# Autodesk Inventor assembly: Rover
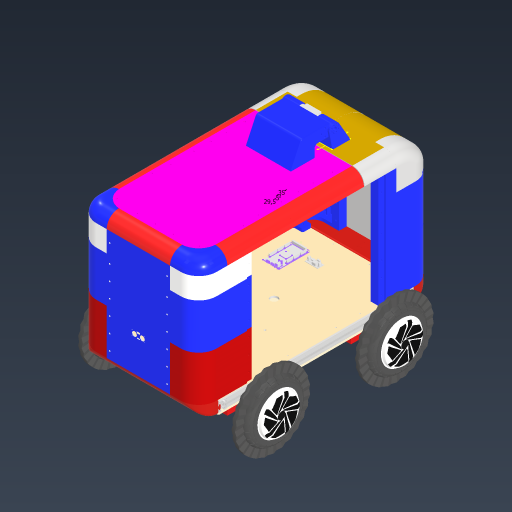
[picture p0: Inventor's stored thumbnail of the model, 512x512]
Saved by Autodesk Inventor 2023.2 (Build 272271030, 271C)
## iProperties
Created: 2024-10-30
Part Number: Rover
Document SubType Name: Assembly
Designer: I9232
Author: I9232
## Documents named in this file (30)
- D:\!Rover\Rover\Rover_construction\Rover.iam
- D:\!Rover\Rover\Rover_construction\platform.ipt
- D:\!Rover\Rover\Rover_construction\Motor, BLDC, Hoverboard Wheel, 8.0in.ipt
- D:\!Rover\Rover\Rover_construction\Profil 20x20.ipt
- D:\!Rover\Rover\Rover_construction\Крепление мотора.iam
- D:\!Rover\Rover\Rover_construction\Уголок для профиля.ipt
- D:\!Rover\Rover\Rover_construction\Профиль 30x30\Профиль 30x30.ipt
- D:\!Rover\Rover\Rover_construction\Т-образный соединитель\Т-образный соединитель.ipt
- D:\!Rover\Rover\Rover_construction\Подъёмник.iam
- D:\!Rover\Rover\Rover_construction\Боковая часть корпуса.ipt
- D:\!Rover\Rover\Rover_construction\Передняя_Задняя фанера.ipt
- D:\!Rover\Rover\Rover_construction\Столбик.ipt
- D:\!Rover\Rover\Rover_construction\Крышка.ipt
- D:\!Rover\Rover\Rover_construction\Вторая часть петли.ipt
- D:\!Rover\Rover\Rover_construction\рдс150.ipt
- D:\!Rover\Rover\Rover_construction\Arduino_Due\Arduino_Due.ipt
- D:\!Rover\Rover\Rover_construction\LM2596 DC-DC stepdown voltage converter\LM2596 DC-DC stepdown voltage converter.ipt
- D:\!Rover\Rover\Rover_construction\DS51_Arm_Disc\DS51_Arm_Disc.ipt
- D:\!Rover\Rover\Rover_construction\Крепление датчика ульразвука.iam
- D:\!Rover\Rover\Rover_construction\Нижний край корпуса.ipt
- D:\!Rover\Rover\Rover_construction\Задний_столб.iam
- D:\!Rover\Rover\Rover_construction\Столб_переда_корпуса_2.0.iam
- D:\!Rover\Rover\Rover_construction\2.0_Ушко петли крышки.ipt
- D:\!Rover\Rover\Rover_construction\2.0_Ушко петли крышки_MIR.ipt
- D:\!Rover\Rover\Rover_construction\2.0_Уголок_передней_крышки.ipt
- D:\!Rover\Rover\Rover_construction\2.0_Уголок_передней_крышки_MIR.ipt
- D:\!Rover\Rover\Rover_construction\2.0_передняя_фанера.ipt
- D:\!Rover\Rover\Rover_construction\Столб_переда_корпуса_2.0_MIR1.iam
- D:\!Rover\Rover\Rover_construction\Задний_столб_MIR1.iam
- D:\!Rover\Rover\Rover_construction\Крышка.iam
## Components (51 placed, 29 different names)
1. platform:1 — Совмещение:1, Совмещение:2, Совмещение:169, Заподлицо:1, Заподлицо:2, Совмещение:170, Совмещение:171, Совмещение:172, Заподлицо:3, Заподлицо:4, Заподлицо:5, Заподлицо:6, Совмещение:180, Заподлицо:11, Совмещение:189, Заподлицо:24, Заподлицо:25, Совмещение:190, Заподлицо:26, Заподлицо:27, Заподлицо:28, Совмещение:191, Заподлицо:29, Совмещение:192, Заподлицо:30, Заподлицо:31, Заподлицо:37, Заподлицо:63
2. Т-образный соединитель:1 — Заподлицо:21, Совмещение:188
3. Т-образный соединитель:2 — Совмещение:187, Заподлицо:23
4. Подъёмник:1 [sub-assembly] — Совмещение:355, Совмещение:356
5. platform:2 — Заподлицо:37, Заподлицо:38, Совмещение:313, Совмещение:314, Совмещение:315, Совмещение:316, Совмещение:317, Заподлицо:46, Заподлицо:47, Совмещение:350, Совмещение:351, Совмещение:355, Заподлицо:62, Заподлицо:72
6. Боковая часть корпуса:1 — Симметрия:4
7. Боковая часть корпуса:2 — Симметрия:4
8. Передняя_Задняя фанера:2 — Совмещение:445, Совмещение:446, Совмещение:447, Совмещение:450
9. Столбик:2 — Совмещение:329, Заподлицо:46, Заподлицо:47
10. Крышка:1 — Совмещение:418, Заподлицо:70, Совмещение:421, Совмещение:424, Совмещение:429, Совмещение:430, Заподлицо:71, Совмещение:432, Совмещение:433, Совмещение:438
11. Вторая часть петли:2 — Совмещение:451, Заподлицо:73, Совмещение:452, Совмещение:453, Совмещение:455
12. рдс150:1 — Совмещение:452, Совмещение:453, Совмещение:454, Совмещение:455
13. Arduino_Due:1 — Совмещение:350, Совмещение:354
14. LM2596 DC-DC stepdown voltage converter:1 — Совмещение:351, Совмещение:354
15. DS51_Arm_Disc:1 — Цилиндрический:1, Совмещение:422, Совмещение:423, Совмещение:454
16. DS51_Arm_Disc:2 — Совмещение:425, Совмещение:426, Цилиндрический:2
17. Крепление датчика ульразвука:1 [sub-assembly]
18. Нижний край корпуса:1 — Совмещение:376, Заподлицо:59, Совмещение:437, Совмещение:442, Совмещение:443, Совмещение:444, Совмещение:447
19. Нижний край корпуса:2 — Совмещение:377, Заподлицо:61, Совмещение:419, Совмещение:436, Совмещение:440
20. Задний_столб:1 [sub-assembly] — Совмещение:381, Заподлицо:63, Совмещение:437, Совмещение:444, Совмещение:445, Совмещение:446, Совмещение:448, Совмещение:449
21. Столб_переда_корпуса_2.0:1 [sub-assembly] — Заподлицо:62, Совмещение:380, Совмещение:418, Заподлицо:70, Совмещение:419, Совмещение:431, Совмещение:434, Совмещение:435
22. 2.0_Ушко петли крышки:1 — Совмещение:421, Цилиндрический:1, Совмещение:422, Совмещение:423, Совмещение:438
23. 2.0_Ушко петли крышки_MIR:1 — Совмещение:424, Совмещение:425, Совмещение:426, Цилиндрический:2
24. 2.0_Уголок_передней_крышки:1 — Совмещение:429, Совмещение:430, Заподлицо:71
25. 2.0_Уголок_передней_крышки_MIR:1 — Совмещение:431, Совмещение:432, Совмещение:433
26. 2.0_передняя_фанера:1 — Совмещение:434, Совмещение:435, Совмещение:436
27. Столб_переда_корпуса_2.0_MIR1:1 [sub-assembly] — Совмещение:439, Совмещение:440, Заподлицо:72
28. Задний_столб_MIR1:1 [sub-assembly] — Совмещение:441, Совмещение:442, Совмещение:443
29. Крепление датчика ульразвука:2 [sub-assembly]
30. Крепление датчика ульразвука:3 [sub-assembly]
31. Крышка:2 [sub-assembly] — Совмещение:448, Совмещение:449, Совмещение:450, Совмещение:451, Заподлицо:73
32. Мотор гироскутера — Совмещение:196, Совмещение:197, Совмещение:198
33. Motor, BLDC, Hoverboard Wheel, 8.0in:4 — Совмещение:199, Совмещение:200, Совмещение:201
34. Motor, BLDC, Hoverboard Wheel, 8.0in:5 — Совмещение:193, Совмещение:194, Совмещение:195
35. Motor, BLDC, Hoverboard Wheel, 8.0in:6 — Совмещение:202, Совмещение:203, Совмещение:204
36. Profil 20x20:1 — Симметрия:3, Заподлицо:14, Совмещение:184, Заподлицо:18
37. Profil 20x20:2 — Симметрия:3, Заподлицо:12, Совмещение:181, Заподлицо:13
38. Profil 20x20:3 — Заподлицо:18
39. Профиль 30x30:5 — Совмещение:179, Совмещение:180, Заподлицо:11, Заподлицо:21, Заподлицо:23
40. Профиль 30x30:2 — Совмещение:171, Совмещение:173, Заподлицо:3, Заподлицо:7, Заподлицо:12, Совмещение:181, Заподлицо:35, Заподлицо:38
41. Профиль 30x30:3 — Совмещение:170, Заподлицо:5, Заподлицо:6, Совмещение:188, Совмещение:313, Совмещение:371, Совмещение:372, Совмещение:377, Заподлицо:61
42. Профиль 30x30:4 — Совмещение:172, Совмещение:174, Заподлицо:4, Совмещение:178, Заподлицо:13, Заподлицо:14, Совмещение:184, Совмещение:219
43. Профиль 30x30:1 — Совмещение:169, Заподлицо:1, Заподлицо:2, Совмещение:173, Совмещение:174, Совмещение:179, Совмещение:187, Заподлицо:55, Заподлицо:56, Совмещение:376, Заподлицо:59
44. Крепление мотора:1 [sub-assembly] — Совмещение:189, Заподлицо:24, Заподлицо:25, Совмещение:199, Совмещение:200, Совмещение:201
45. Крепление мотора:2 [sub-assembly] — Совмещение:190, Заподлицо:26, Заподлицо:27, Совмещение:196, Совмещение:197, Совмещение:198
46. Крепление мотора:3 [sub-assembly] — Заподлицо:28, Совмещение:191, Заподлицо:29, Совмещение:202, Совмещение:203, Совмещение:204
47. Крепление мотора:4 [sub-assembly] — Совмещение:192, Заподлицо:30, Заподлицо:31, Совмещение:193, Совмещение:194, Совмещение:195
48. Уголок для профиля:1 — Совмещение:178, Совмещение:317, Заподлицо:55, Совмещение:381
49. Уголок для профиля:2 — Заподлицо:7, Совмещение:314, Совмещение:371, Совмещение:380
50. Уголок для профиля:3 — Заподлицо:35, Совмещение:316, Заподлицо:56, Совмещение:441
51. Уголок для профиля:4 — Совмещение:219, Совмещение:315, Совмещение:329, Совмещение:372, Совмещение:439
## Relationships (125: Mate 84, Flush 37, Symmetry 2, CylindricalJoint 2)
- Совмещение:1 [Mate]: platform:1
- Совмещение:2 [Mate]: platform:1
- Симметрия:3 [Symmetry]: Profil 20x20:1 ↔ Profil 20x20:2
- Совмещение:169 [Mate]: platform:1 ↔ Профиль 30x30:1
- Заподлицо:1 [Flush]: platform:1 ↔ Профиль 30x30:1
- Заподлицо:2 [Flush]: platform:1 ↔ Профиль 30x30:1
- Совмещение:170 [Mate]: platform:1 ↔ Профиль 30x30:3
- Совмещение:171 [Mate]: platform:1 ↔ Профиль 30x30:2
- Совмещение:172 [Mate]: platform:1 ↔ Профиль 30x30:4
- Совмещение:173 [Mate]: Профиль 30x30:2 ↔ Профиль 30x30:1
- Заподлицо:3 [Flush]: platform:1 ↔ Профиль 30x30:2
- Совмещение:174 [Mate]: Профиль 30x30:4 ↔ Профиль 30x30:1
- Заподлицо:4 [Flush]: platform:1 ↔ Профиль 30x30:4
- Заподлицо:5 [Flush]: platform:1 ↔ Профиль 30x30:3
- Заподлицо:6 [Flush]: platform:1 ↔ Профиль 30x30:3
- Заподлицо:7 [Flush]: Профиль 30x30:2 ↔ Уголок для профиля:2
- Совмещение:178 [Mate]: Профиль 30x30:4 ↔ Уголок для профиля:1
- Совмещение:179 [Mate]: Профиль 30x30:5 ↔ Профиль 30x30:1
- Совмещение:180 [Mate]: platform:1 ↔ Профиль 30x30:5
- Заподлицо:11 [Flush]: platform:1 ↔ Профиль 30x30:5
- Заподлицо:12 [Flush]: Profil 20x20:2 ↔ Профиль 30x30:2
- Совмещение:181 [Mate]: Profil 20x20:2 ↔ Профиль 30x30:2
- Заподлицо:13 [Flush]: Profil 20x20:2 ↔ Профиль 30x30:4
- Заподлицо:14 [Flush]: Profil 20x20:1 ↔ Профиль 30x30:4
- Совмещение:184 [Mate]: Profil 20x20:1 ↔ Профиль 30x30:4
- Заподлицо:18 [Flush] (-200 mm): Profil 20x20:1 ↔ Profil 20x20:3
- Заподлицо:21 [Flush]: Т-образный соединитель:1 ↔ Профиль 30x30:5
- Совмещение:187 [Mate]: Т-образный соединитель:2 ↔ Профиль 30x30:1
- Заподлицо:23 [Flush]: Т-образный соединитель:2 ↔ Профиль 30x30:5
- Совмещение:188 [Mate]: Т-образный соединитель:1 ↔ Профиль 30x30:3
- Совмещение:189 [Mate]: platform:1 ↔ Крепление мотора:1
- Заподлицо:24 [Flush] (30 mm): platform:1 ↔ Крепление мотора:1
- Заподлицо:25 [Flush]: platform:1 ↔ Крепление мотора:1
- Совмещение:190 [Mate]: platform:1 ↔ Крепление мотора:2
- Заподлицо:26 [Flush] (30 mm): platform:1 ↔ Крепление мотора:2
- Заподлицо:27 [Flush]: platform:1 ↔ Крепление мотора:2
- Заподлицо:28 [Flush] (30 mm): platform:1 ↔ Крепление мотора:3
- Совмещение:191 [Mate]: platform:1 ↔ Крепление мотора:3
- Заподлицо:29 [Flush]: platform:1 ↔ Крепление мотора:3
- Совмещение:192 [Mate]: platform:1 ↔ Крепление мотора:4
- Заподлицо:30 [Flush]: platform:1 ↔ Крепление мотора:4
- Заподлицо:31 [Flush] (30 mm): platform:1 ↔ Крепление мотора:4
- Совмещение:193 [Mate]: Motor, BLDC, Hoverboard Wheel, 8.0in:5 ↔ Крепление мотора:4
- Совмещение:194 [Mate]: Motor, BLDC, Hoverboard Wheel, 8.0in:5 ↔ Крепление мотора:4
- Совмещение:195 [Mate]: Motor, BLDC, Hoverboard Wheel, 8.0in:5 ↔ Крепление мотора:4
- Совмещение:196 [Mate]: Мотор гироскутера ↔ Крепление мотора:2
- Совмещение:197 [Mate]: Мотор гироскутера ↔ Крепление мотора:2
- Совмещение:198 [Mate]: Мотор гироскутера ↔ Крепление мотора:2
- Совмещение:199 [Mate]: Motor, BLDC, Hoverboard Wheel, 8.0in:4 ↔ Крепление мотора:1
- Совмещение:200 [Mate]: Motor, BLDC, Hoverboard Wheel, 8.0in:4 ↔ Крепление мотора:1
- Совмещение:201 [Mate]: Motor, BLDC, Hoverboard Wheel, 8.0in:4 ↔ Крепление мотора:1
- Совмещение:202 [Mate]: Motor, BLDC, Hoverboard Wheel, 8.0in:6 ↔ Крепление мотора:3
- Совмещение:203 [Mate]: Motor, BLDC, Hoverboard Wheel, 8.0in:6 ↔ Крепление мотора:3
- Совмещение:204 [Mate]: Motor, BLDC, Hoverboard Wheel, 8.0in:6 ↔ Крепление мотора:3
- Совмещение:219 [Mate]: Профиль 30x30:4 ↔ Уголок для профиля:4
- Заподлицо:35 [Flush]: Профиль 30x30:2 ↔ Уголок для профиля:3
- Заподлицо:37 [Flush]: platform:1 ↔ platform:2
- Заподлицо:38 [Flush]: platform:2 ↔ Профиль 30x30:2
- Совмещение:313 [Mate]: platform:2 ↔ Профиль 30x30:3
- Совмещение:314 [Mate]: platform:2 ↔ Уголок для профиля:2
- Совмещение:315 [Mate]: platform:2 ↔ Уголок для профиля:4
- Совмещение:316 [Mate]: platform:2 ↔ Уголок для профиля:3
- Совмещение:317 [Mate]: platform:2 ↔ Уголок для профиля:1
- Симметрия:4 [Symmetry]: Боковая часть корпуса:1 ↔ Боковая часть корпуса:2
- Совмещение:329 [Mate]: Столбик:2 ↔ Уголок для профиля:4
- Заподлицо:46 [Flush]: platform:2 ↔ Столбик:2
- Заподлицо:47 [Flush]: platform:2 ↔ Столбик:2
- Совмещение:350 [Mate]: platform:2 ↔ Arduino_Due:1
- Совмещение:351 [Mate]: platform:2 ↔ LM2596 DC-DC stepdown voltage converter:1
- Совмещение:354 [Mate] (20 mm): Arduino_Due:1 ↔ LM2596 DC-DC stepdown voltage converter:1
- Совмещение:355 [Mate]: Подъёмник:1 ↔ platform:2
- Совмещение:356 [Mate]: Подъёмник:1
- Совмещение:371 [Mate]: Профиль 30x30:3 ↔ Уголок для профиля:2
- Заподлицо:55 [Flush]: Профиль 30x30:1 ↔ Уголок для профиля:1
- Совмещение:372 [Mate]: Профиль 30x30:3 ↔ Уголок для профиля:4
- Заподлицо:56 [Flush]: Профиль 30x30:1 ↔ Уголок для профиля:3
- Совмещение:376 [Mate]: Нижний край корпуса:1 ↔ Профиль 30x30:1
- Заподлицо:59 [Flush]: Нижний край корпуса:1 ↔ Профиль 30x30:1
- Совмещение:377 [Mate]: Нижний край корпуса:2 ↔ Профиль 30x30:3
- Заподлицо:61 [Flush]: Нижний край корпуса:2 ↔ Профиль 30x30:3
- Заподлицо:62 [Flush]: platform:2 ↔ Столб_переда_корпуса_2.0:1
- Совмещение:380 [Mate]: Столб_переда_корпуса_2.0:1 ↔ Уголок для профиля:2
- Совмещение:381 [Mate]: Задний_столб:1 ↔ Уголок для профиля:1
- Заподлицо:63 [Flush]: platform:1 ↔ Задний_столб:1
- Совмещение:418 [Mate]: Крышка:1 ↔ Столб_переда_корпуса_2.0:1
- Заподлицо:70 [Flush]: Крышка:1 ↔ Столб_переда_корпуса_2.0:1
- Совмещение:419 [Mate]: Нижний край корпуса:2 ↔ Столб_переда_корпуса_2.0:1
- Совмещение:421 [Mate]: Крышка:1 ↔ 2.0_Ушко петли крышки:1
- Цилиндрический:1 [CylindricalJoint]: DS51_Arm_Disc:1 ↔ 2.0_Ушко петли крышки:1
- Совмещение:422 [Mate]: DS51_Arm_Disc:1 ↔ 2.0_Ушко петли крышки:1
- Совмещение:423 [Mate] (1 mm): DS51_Arm_Disc:1 ↔ 2.0_Ушко петли крышки:1
- Совмещение:424 [Mate]: Крышка:1 ↔ 2.0_Ушко петли крышки_MIR:1
- Совмещение:425 [Mate] (1 mm): DS51_Arm_Disc:2 ↔ 2.0_Ушко петли крышки_MIR:1
- Совмещение:426 [Mate]: DS51_Arm_Disc:2 ↔ 2.0_Ушко петли крышки_MIR:1
- Цилиндрический:2 [CylindricalJoint]: DS51_Arm_Disc:2 ↔ 2.0_Ушко петли крышки_MIR:1
- Совмещение:429 [Mate]: Крышка:1 ↔ 2.0_Уголок_передней_крышки:1
- Совмещение:430 [Mate]: Крышка:1 ↔ 2.0_Уголок_передней_крышки:1
- Заподлицо:71 [Flush]: Крышка:1 ↔ 2.0_Уголок_передней_крышки:1
- Совмещение:431 [Mate]: Столб_переда_корпуса_2.0:1 ↔ 2.0_Уголок_передней_крышки_MIR:1
- Совмещение:432 [Mate]: Крышка:1 ↔ 2.0_Уголок_передней_крышки_MIR:1
- Совмещение:433 [Mate]: Крышка:1 ↔ 2.0_Уголок_передней_крышки_MIR:1
- Совмещение:434 [Mate]: Столб_переда_корпуса_2.0:1 ↔ 2.0_передняя_фанера:1
- Совмещение:435 [Mate]: Столб_переда_корпуса_2.0:1 ↔ 2.0_передняя_фанера:1
- Совмещение:436 [Mate]: Нижний край корпуса:2 ↔ 2.0_передняя_фанера:1
- Совмещение:437 [Mate]: Нижний край корпуса:1 ↔ Задний_столб:1
- Совмещение:438 [Mate] (1 mm): Крышка:1 ↔ 2.0_Ушко петли крышки:1
- Совмещение:439 [Mate]: Столб_переда_корпуса_2.0_MIR1:1 ↔ Уголок для профиля:4
- Совмещение:440 [Mate]: Нижний край корпуса:2 ↔ Столб_переда_корпуса_2.0_MIR1:1
- Заподлицо:72 [Flush]: platform:2 ↔ Столб_переда_корпуса_2.0_MIR1:1
- Совмещение:441 [Mate]: Задний_столб_MIR1:1 ↔ Уголок для профиля:3
- Совмещение:442 [Mate]: Нижний край корпуса:1 ↔ Задний_столб_MIR1:1
- Совмещение:443 [Mate]: Нижний край корпуса:1 ↔ Задний_столб_MIR1:1
- Совмещение:444 [Mate]: Нижний край корпуса:1 ↔ Задний_столб:1
- Совмещение:445 [Mate]: Передняя_Задняя фанера:2 ↔ Задний_столб:1
- Совмещение:446 [Mate]: Передняя_Задняя фанера:2 ↔ Задний_столб:1
- Совмещение:447 [Mate]: Передняя_Задняя фанера:2 ↔ Нижний край корпуса:1
- Совмещение:448 [Mate]: Задний_столб:1 ↔ Крышка:2
- Совмещение:449 [Mate]: Задний_столб:1 ↔ Крышка:2
- Совмещение:450 [Mate]: Передняя_Задняя фанера:2 ↔ Крышка:2
- Совмещение:451 [Mate]: Вторая часть петли:2 ↔ Крышка:2
- Заподлицо:73 [Flush]: Вторая часть петли:2 ↔ Крышка:2
- Совмещение:452 [Mate]: Вторая часть петли:2 ↔ рдс150:1
- Совмещение:453 [Mate] (0.5 mm): Вторая часть петли:2 ↔ рдс150:1
- Совмещение:454 [Mate]: рдс150:1 ↔ DS51_Arm_Disc:1
- Совмещение:455 [Mate] (0.5 mm): Вторая часть петли:2 ↔ рдс150:1
